# Autodesk Inventor assembly: Assembly_Micromanipulator
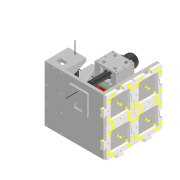
[picture p0: Inventor's stored thumbnail of the model, 180x180]
Saved by Autodesk Inventor 2022 (Build 260153000, 153)
## iProperties
Created: 2022-12-17
Part Number: Assembly_Micromanipulator
Document SubType Name: Assembly
Designer: diederichbenedict
Author: diederichbenedict
## Documents named in this file (4)
- C:\Users\diederichbenedict\Dropbox\Dokumente\Promotion\PROJECTS\openUC2-CAD\INVENTOR\Assembly_Micromanipulator.iam
- C:\Users\diederichbenedict\Dropbox\Dokumente\Promotion\PROJECTS\openUC2-CAD\INVENTOR\Assembly_Linear_MGN8_Noncaptive.iam
- C:\Users\diederichbenedict\Dropbox\Dokumente\Promotion\PROJECTS\openUC2-CAD\INVENTOR\30_Linear_Captive_Nema8_Stand.ipt
- C:\Users\diederichbenedict\Dropbox\Dokumente\Promotion\PROJECTS\openUC2-CAD\INVENTOR\10_Base_puzzle_v3.ipt
## Components (8 placed, 3 different names)
1. Assembly_Linear_MGN8_Noncaptive:1 [sub-assembly] — Fluchtend:1, Passend:3, Fluchtend:3, Fluchtend:5, Fluchtend:6
2. Assembly_Linear_MGN8_Noncaptive:2 [sub-assembly] — Fluchtend:1, Passend:2, Fluchtend:2, Passend:3, Fluchtend:3, Fluchtend:4
3. Assembly_Linear_MGN8_Noncaptive:3 [sub-assembly] — Passend:2, Fluchtend:2, Fluchtend:4
4. 30_Linear_Captive_Nema8_Stand:1 — Fluchtend:5, Fluchtend:6, Passend:4, Fluchtend:7, Fluchtend:8
5. 10_Base_puzzle_v3:1
6. 10_Base_puzzle_v3:2
7. 10_Base_puzzle_v3:3 — Passend:4, Fluchtend:7
8. 10_Base_puzzle_v3:4 — Fluchtend:8
## Component patterns: (4 elements, first: 10_Base_puzzle_v3:1)
## Relationships (11: Flush 8, Mate 3)
- Fluchtend:1 [Flush]: Assembly_Linear_MGN8_Noncaptive:1 ↔ Assembly_Linear_MGN8_Noncaptive:2
- Passend:2 [Mate]: Assembly_Linear_MGN8_Noncaptive:2 ↔ Assembly_Linear_MGN8_Noncaptive:3
- Fluchtend:2 [Flush]: Assembly_Linear_MGN8_Noncaptive:2 ↔ Assembly_Linear_MGN8_Noncaptive:3
- Passend:3 [Mate]: Assembly_Linear_MGN8_Noncaptive:1 ↔ Assembly_Linear_MGN8_Noncaptive:2
- Fluchtend:3 [Flush]: Assembly_Linear_MGN8_Noncaptive:1 ↔ Assembly_Linear_MGN8_Noncaptive:2
- Fluchtend:4 [Flush]: Assembly_Linear_MGN8_Noncaptive:2 ↔ Assembly_Linear_MGN8_Noncaptive:3
- Fluchtend:5 [Flush]: Assembly_Linear_MGN8_Noncaptive:1 ↔ 30_Linear_Captive_Nema8_Stand:1
- Fluchtend:6 [Flush]: Assembly_Linear_MGN8_Noncaptive:1 ↔ 30_Linear_Captive_Nema8_Stand:1
- Passend:4 [Mate]: 30_Linear_Captive_Nema8_Stand:1 ↔ 10_Base_puzzle_v3:3
- Fluchtend:7 [Flush]: 30_Linear_Captive_Nema8_Stand:1 ↔ 10_Base_puzzle_v3:3
- Fluchtend:8 [Flush]: 30_Linear_Captive_Nema8_Stand:1 ↔ 10_Base_puzzle_v3:4
